# Autodesk Inventor assembly: Shoulder V2
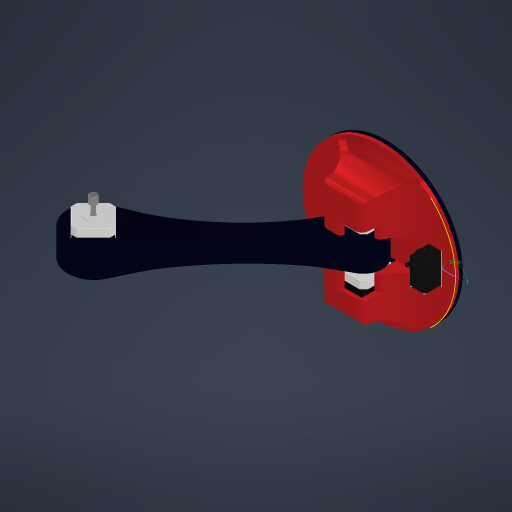
[picture p0: Inventor's stored thumbnail of the model, 512x512]
Saved by Autodesk Inventor 2023 (Build 270158000, 158)
## iProperties
Created: 2023-04-08
Part Number: Shoulder V2
Document SubType Name: Assembly
Designer: vatdu
Author: vatdu
## Documents named in this file (6)
- C:\Users\vatdu\Desktop\CRYSTAL MARK II\Arm\Shoulder\Shoulder V2.iam
- C:\Users\vatdu\Desktop\CRYSTAL MARK II\Components\Stepper Motor.ipt
- C:\Users\vatdu\Desktop\CRYSTAL MARK II\Arm\Shoulder\Rotating Plate.ipt
- C:\Users\vatdu\Desktop\CRYSTAL MARK II\Arm\Shoulder\Motor Cover V2.ipt
- C:\Users\vatdu\Desktop\CRYSTAL MARK II\Arm\Shoulder\Arm.ipt
- C:\Users\vatdu\Desktop\CRYSTAL MARK II\Components\Servo.ipt
## Components (7 placed, 5 different names)
1. Stepper Motor:1 — Rigid:3
2. Stepper Motor:2 — Rigid:4, Rigid:6
3. Stepper Motor:3 — Rigid:1, Rotational:2, Rigid:5
4. Rotating Plate:1 — Rotational:1
5. Motor Cover V2:1 — Rigid:1, Rigid:3, Rotational:1
6. Arm:1 — Rigid:4, Rotational:2, Rigid:5, Rigid:6
7. Servo:1
## Relationships (7: WeldJoint 5, RevoluteJoint 2)
- Rigid:1 [WeldJoint]: Stepper Motor:3 ↔ Motor Cover V2:1
- Rigid:3 [WeldJoint]: Stepper Motor:1 ↔ Motor Cover V2:1
- Rotational:1 [RevoluteJoint]: Rotating Plate:1 ↔ Motor Cover V2:1
- Rigid:4 [WeldJoint]: Stepper Motor:2 ↔ Arm:1
- Rotational:2 [RevoluteJoint] (-8.05 mm): Stepper Motor:3 ↔ Arm:1
- Rigid:5 [WeldJoint] (-1 mm): Stepper Motor:3 ↔ Arm:1
- Rigid:6 [WeldJoint]: Stepper Motor:2 ↔ Arm:1
